# Autodesk Inventor assembly: rightSide
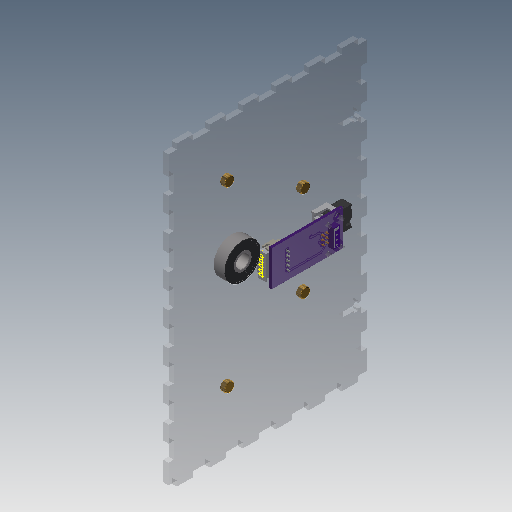
[picture p0: Inventor's stored thumbnail of the model, 512x512]
Saved by Autodesk Inventor 2018 (Build 220112000, 112)
## iProperties
Created: 2016-08-27
Part Number: rightSide
Document SubType Name: Assembly
Designer: sawaiz
Author: sawaiz
## Documents named in this file (6)
- C:\Users\sawaiz\OneDrive\projects\splitFlapDisplay\frame\rightSide.iam
- C:\Users\sawaiz\OneDrive\projects\splitFlapDisplay\frame\rightSide.ipt
- C:\Users\sawaiz\OneDrive\projects\splitFlapDisplay\frame\magnet.ipt
- C:\Users\sawaiz\OneDrive\projects\splitFlapDisplay\frame\608RS.ipt
- C:\Users\sawaiz\OneDrive\projects\splitFlapDisplay\electronics\cad\landing\landing.ipt
- C:\Users\sawaiz\OneDrive\projects\splitFlapDisplay\electronics\cad\uC\uC.iam
## Components (9 placed, 5 different names)
1. rightSide:1 — Flush:4, Mate:1, Mate:2, Mate:3, Mate:4, Mate:5, Flush:5, Mate:7, Mate:8, Mate:9, Angle:1, Mate:11, Mate:12
2. magnet:1 — Flush:1, Mate:4
3. magnet:2 — Flush:1, Flush:2, Mate:3
4. magnet:3 — Flush:2, Flush:3, Mate:2
5. magnet:4 — Flush:3, Flush:4, Mate:1
6. 608RS:1 — Mate:5, Flush:5
7. landing:1 — Flush:6, Flush:7, Mate:6, Mate:10
8. landing:2 — Flush:6, Flush:7, Mate:6, Angle:1, Mate:11, Mate:12
9. uC:1 [sub-assembly] — Mate:7, Mate:8, Mate:9, Mate:10
## Relationships (20: Mate 12, Flush 7, Angle 1)
- Flush:1: magnet:1 ↔ magnet:2
- Flush:2: magnet:2 ↔ magnet:3
- Flush:3: magnet:3 ↔ magnet:4
- Flush:4: rightSide:1 ↔ magnet:4
- Mate:1: rightSide:1 ↔ magnet:4
- Mate:2: rightSide:1 ↔ magnet:3
- Mate:3: rightSide:1 ↔ magnet:2
- Mate:4: rightSide:1 ↔ magnet:1
- Mate:5: rightSide:1 ↔ 608RS:1
- Flush:5: rightSide:1 ↔ 608RS:1
- Flush:6: landing:1 ↔ landing:2
- Flush:7: landing:1 ↔ landing:2
- Mate:6: landing:1 ↔ landing:2
- Mate:7: rightSide:1 ↔ uC:1
- Mate:8: rightSide:1 ↔ uC:1
- Mate:9: rightSide:1 ↔ uC:1
- Mate:10: landing:1 ↔ uC:1
- Angle:1 (0 deg): rightSide:1 ↔ landing:2
- Mate:11: rightSide:1 ↔ landing:2
- Mate:12: rightSide:1 ↔ landing:2
